# Autodesk Inventor assembly: mounted servo
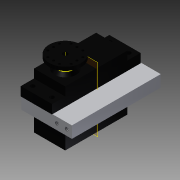
[picture p0: Inventor's stored thumbnail of the model, 180x180]
Saved by Autodesk Inventor 2013 (Build 170138000, 138)
## iProperties
Created: 2013-09-17
Part Number: mounted servo
Document SubType Name: Assembly
Designer: Ian
Author: Ian
## Documents named in this file (3)
- C:\Users\Ian\Documents\Inventor\xyPartStorage\mounted servo.iam
- C:\Users\Ian\Documents\Inventor\xyPartStorage\stepper\servo_mount.ipt
- C:\Users\Ian\Documents\Inventor\xyPartStorage\servo-dummy\servo-dummy.iam
## Components (2 placed, 2 different names)
1. servo_mount:1 — Mate:1, Mate:2, Mate:3
2. servo-dummy:1 [sub-assembly] — Mate:1, Mate:2, Mate:3
## Relationships (3: Mate 3)
- Mate:1: servo_mount:1 ↔ servo-dummy:1
- Mate:2: servo_mount:1 ↔ servo-dummy:1
- Mate:3: servo_mount:1 ↔ servo-dummy:1
